# Autodesk Inventor assembly: CuttingHead
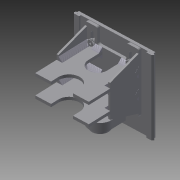
[picture p0: Inventor's stored thumbnail of the model, 180x180]
Saved by Autodesk Inventor 2013 (Build 170138000, 138)
## iProperties
Created: 2012-12-07
Part Number: CuttingHead
Document SubType Name: Assembly
Designer: istvan.burbank
Mass: 179.257 g
Surface Area: 890.164 cm^2
Volume: 179.257 cm^3
Density: 1 g/cm^3
Author: istvan.burbank
## Documents named in this file (8)
- E:\GitHub\Crown-Fire\CAD\CuttingHead\CuttingHead.iam
- E:\GitHub\Crown-Fire\CAD\CuttingHead\AcmeRoundNut.ipt
- E:\GitHub\Crown-Fire\CAD\CuttingHead\AcmeMountingFlange.ipt
- E:\GitHub\Crown-Fire\CAD\CuttingHead\backPlate.ipt
- E:\GitHub\Crown-Fire\CAD\Hardware\z-axisSliderShoulderBolts.ipt
- E:\GitHub\Crown-Fire\CAD\CuttingHead\torchArm.iam
- E:\GitHub\Crown-Fire\CAD\CuttingHead\z-vee-track.ipt
- E:\GitHub\Crown-Fire\CAD\Templates\vee-track.ipt
## Components (10 placed, 6 different names)
1. AcmeRoundNut:1 — Mate:1, Mate:2
2. AcmeMountingFlange:1 — Mate:1, Mate:2, Mate:3, Flush:3
3. backPlate:1 — Mate:3, Flush:3, Mate:8, Mate:9, Mate:10, Mate:11, Mate:12, Mate:13, Mate:14, Flush:4, Flush:5, Mate:15, Mate:16
4. z-axisSliderShoulderBolts:1 — Mate:8, Tangent:1
5. z-axisSliderShoulderBolts:2 — Mate:9, Tangent:3
6. z-axisSliderShoulderBolts:3 — Mate:10, Tangent:2
7. z-axisSliderShoulderBolts:4 — Mate:11, Tangent:4
8. torchArm:1 [sub-assembly] — Tangent:1, Tangent:2, Tangent:3, Tangent:4, Mate:12
9. z-vee-track:1 — Mate:14, Flush:5, Mate:16
10. z-vee-track:2 — Mate:13, Flush:4, Mate:15
## Relationships (19: Mate 12, Tangent 4, Flush 3)
- Mate:1: AcmeRoundNut:1 ↔ AcmeMountingFlange:1
- Mate:2: AcmeRoundNut:1 ↔ AcmeMountingFlange:1
- Mate:3: AcmeMountingFlange:1 ↔ backPlate:1
- Flush:3 (-6.35 mm): AcmeMountingFlange:1 ↔ backPlate:1
- Mate:8: backPlate:1 ↔ z-axisSliderShoulderBolts:1
- Mate:9: backPlate:1 ↔ z-axisSliderShoulderBolts:2
- Mate:10: backPlate:1 ↔ z-axisSliderShoulderBolts:3
- Mate:11: backPlate:1 ↔ z-axisSliderShoulderBolts:4
- Tangent:1: z-axisSliderShoulderBolts:1 ↔ torchArm:1
- Tangent:2: z-axisSliderShoulderBolts:3 ↔ torchArm:1
- Tangent:3: z-axisSliderShoulderBolts:2 ↔ torchArm:1
- Tangent:4: z-axisSliderShoulderBolts:4 ↔ torchArm:1
- Mate:12: backPlate:1 ↔ torchArm:1
- Mate:13: backPlate:1 ↔ z-vee-track:2
- Mate:14: backPlate:1 ↔ z-vee-track:1
- Flush:4: backPlate:1 ↔ z-vee-track:2
- Flush:5: backPlate:1 ↔ z-vee-track:1
- Mate:15: backPlate:1 ↔ z-vee-track:2
- Mate:16: backPlate:1 ↔ z-vee-track:1
